# Autodesk Inventor assembly: derive_road_v14
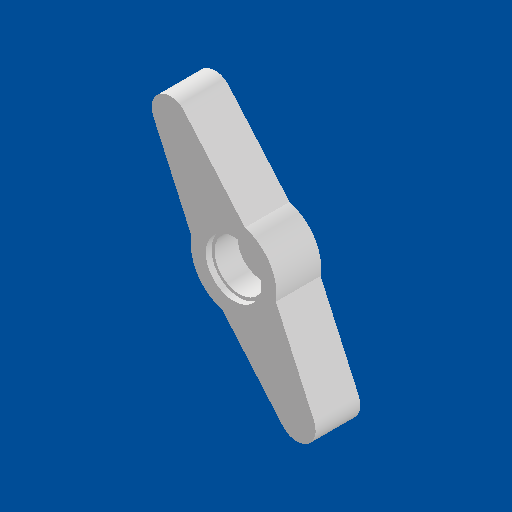
[picture p0: Inventor's stored thumbnail of the model, 512x512]
Saved by Autodesk Inventor 2026.2 (Build 302298000, 298)
## iProperties
Created: 2026-02-24
Part Number: derive_road_v14
Document SubType Name: Assembly
Designer: Thoma
Author: Thoma
## Documents named in this file (3)
- C:\Users\Thoma\OneDrive\Desktop\dir\telescope_cover\cover\derive_rod_v14.iam
- C:\Users\Thoma\OneDrive\Desktop\dir\telescope_cover\cover\rod_v12.ipt
- C:\Users\Thoma\OneDrive\Desktop\dir\telescope_cover\cover\servo_attach.ipt
## Components (2 placed, 2 different names)
1. rod_v12:1 — Flush:1, Mate:1
2. servo_attach:1 — Flush:1, Mate:1
## Relationships (2: Flush 1, Mate 1)
- Flush:1 (1.13 mm): rod_v12:1 ↔ servo_attach:1
- Mate:1: rod_v12:1 ↔ servo_attach:1
